# Autodesk Inventor assembly: main_assy_baraca
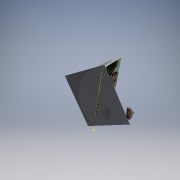
[picture p0: Inventor's stored thumbnail of the model, 180x180]
Saved by Autodesk Inventor 2019 (Build 230136000, 136)
## iProperties
Created: 2019-02-23
Part Number: main_assy_baraca
Document SubType Name: Assembly
Designer: gaincarlo
Author: gaincarlo
## Documents named in this file (13)
- D:\Giancarlo Bacchio\Documenti\00 - Progetti\30-Inventor\LaPanca\main_assy_baraca.iam
- D:\Giancarlo Bacchio\Documenti\00 - Progetti\30-Inventor\LaPanca\concrete_main.ipt
- D:\Giancarlo Bacchio\Documenti\00 - Progetti\30-Inventor\LaPanca\back_plates.iam
- D:\Giancarlo Bacchio\Documenti\00 - Progetti\30-Inventor\LaPanca\back_plates_MIR1.iam
- D:\Giancarlo Bacchio\Documenti\00 - Progetti\30-Inventor\LaPanca\solar_panel.ipt
- D:\Giancarlo Bacchio\Documenti\00 - Progetti\30-Inventor\LaPanca\solar_panel_MIR.ipt
- D:\Giancarlo Bacchio\Documenti\00 - Progetti\30-Inventor\LaPanca\curved-+_plates.iam
- D:\Giancarlo Bacchio\Documenti\00 - Progetti\30-Inventor\LaPanca\curved-+_plates_MIR.iam
- D:\Giancarlo Bacchio\Documenti\00 - Progetti\30-Inventor\LaPanca\table_beam.ipt
- D:\Giancarlo Bacchio\Documenti\00 - Progetti\30-Inventor\LaPanca\support3.ipt
- D:\Giancarlo Bacchio\Documenti\00 - Progetti\30-Inventor\LaPanca\table_beam_MIR1.ipt
- D:\Giancarlo Bacchio\Documenti\00 - Progetti\30-Inventor\LaPanca\doga_long1.ipt
- D:\Giancarlo Bacchio\Documenti\00 - Progetti\30-Inventor\LaPanca\baraca.ipt
## Components (20 placed, 12 different names)
1. concrete_main:1 — Mate:1, Flush:1, Mate:2, Flush:2, Flush:3, Flush:4, Mate:4, Mate:5, Mate:6, Mate:10, Mate:11
2. back_plates:2 [sub-assembly] — Mate:1, Flush:1
3. back_plates_MIR1:1 [sub-assembly]
4. solar_panel:1
5. solar_panel_MIR:1
6. curved-+_plates:1 [sub-assembly] — Mate:3, Flush:4
7. curved-+_plates_MIR:1 [sub-assembly]
8. table_beam:1 — Mate:4, Mate:5, Mate:6, Mate:7, Mate:8
9. table_beam_MIR1:1 — Mate:9, Mate:10, Mate:11
10. baraca:1
11. back_plates:1 [sub-assembly] — Mate:2, Flush:2, Flush:3
12. back_plates:3 [sub-assembly] — Mate:3
13. back_plates_MIR1:2 [sub-assembly]
14. back_plates_MIR1:3 [sub-assembly]
15. support3:1 — Mate:7, Mate:8, Mate:9, Mate:13, Mate:14
16. support3:2 — Mate:12
17. support3:3
18. doga_long1:1 — Mate:12, Mate:13, Mate:14
19. doga_long1:2
20. doga_long1:3
## Component patterns: (2 elements, first: back_plates:1), (2 elements, first: back_plates_MIR1:2), (3 elements, first: support3:1), (3 elements, first: doga_long1:1)
## Relationships (18: Mate 14, Flush 4)
- Mate:1: concrete_main:1 ↔ back_plates:2
- Flush:1 (-25 mm): concrete_main:1 ↔ back_plates:2
- Mate:2: concrete_main:1 ↔ back_plates:1
- Flush:2 (-25 mm): concrete_main:1 ↔ back_plates:1
- Flush:3 (60 mm): concrete_main:1 ↔ back_plates:1
- Mate:3 (25 mm): curved-+_plates:1 ↔ back_plates:3
- Flush:4 (10 mm): concrete_main:1 ↔ curved-+_plates:1
- Mate:4: concrete_main:1 ↔ table_beam:1
- Mate:5: concrete_main:1 ↔ table_beam:1
- Mate:6: concrete_main:1 ↔ table_beam:1
- Mate:7: table_beam:1 ↔ support3:1
- Mate:8: table_beam:1 ↔ support3:1
- Mate:9: table_beam_MIR1:1 ↔ support3:1
- Mate:10: concrete_main:1 ↔ table_beam_MIR1:1
- Mate:11: concrete_main:1 ↔ table_beam_MIR1:1
- Mate:12: support3:2 ↔ doga_long1:1
- Mate:13: support3:1 ↔ doga_long1:1
- Mate:14: support3:1 ↔ doga_long1:1
